# Autodesk Inventor assembly: BASE
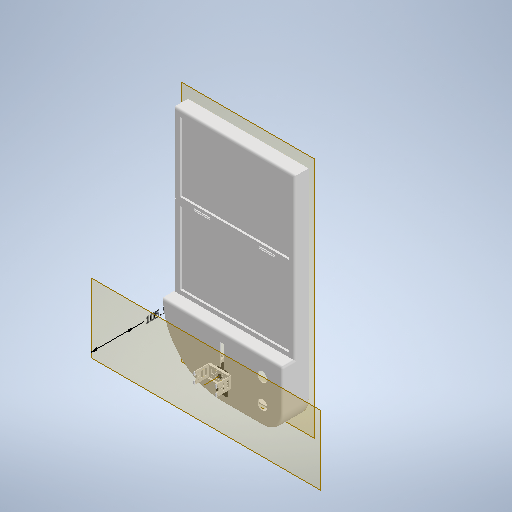
[picture p0: Inventor's stored thumbnail of the model, 512x512]
Saved by Autodesk Inventor 2026.1 (Build 301233020, 233B)
## iProperties
Created: 2025-10-15
Part Number: BASE
Document SubType Name: Assembly
Designer: wlgns
Author: wlgns
## Documents named in this file (5)
- C:\Users\wlgns\Desktop\project\ARA Project\ARA_CAD_model\ARA_v2\BASE.iam
- C:\Users\wlgns\Desktop\project\ARA Project\ARA_CAD_model\ARA_v2\MX-64R.ipt
- C:\Users\wlgns\Desktop\project\ARA Project\ARA_CAD_model\ARA_v2\FR08-H101.ipt
- C:\Users\wlgns\Desktop\project\ARA Project\ARA_CAD_model\ARA_v2\PLATE 1.ipt
- C:\Users\wlgns\Desktop\project\ARA Project\ARA_CAD_model\ARA_v2\PLATE 2.ipt
## Components (4 placed, 4 different names)
1. MX-64R:1 — 메이트:1, 메이트:2, 메이트:5, 메이트:6
2. FR08-H101:1 — 메이트:1, 메이트:2, 플러쉬:1
3. PLATE 1:1 — 메이트:4, 각도:1, 메이트:6, 메이트:7, 메이트:9, 메이트:10, 메이트:11
4. PLATE 2:1 — 메이트:9, 메이트:10, 메이트:11
## Relationships (12: Mate 10, Angle 1, Flush 1)
- 메이트:1 [Mate]: MX-64R:1 ↔ FR08-H101:1
- 메이트:2 [Mate]: MX-64R:1 ↔ FR08-H101:1
- 메이트:4 [Mate]: PLATE 1:1
- 각도:1 [Angle] (0 deg): PLATE 1:1
- 메이트:5 [Mate]: MX-64R:1
- 메이트:6 [Mate]: MX-64R:1 ↔ PLATE 1:1
- 메이트:7 [Mate]: PLATE 1:1
- 메이트:8 [Mate]
- 메이트:9 [Mate]: PLATE 1:1 ↔ PLATE 2:1
- 메이트:10 [Mate]: PLATE 1:1 ↔ PLATE 2:1
- 메이트:11 [Mate]: PLATE 1:1 ↔ PLATE 2:1
- 플러쉬:1 [Flush] (-3 mm): FR08-H101:1
